# Autodesk Inventor assembly: Assembly1
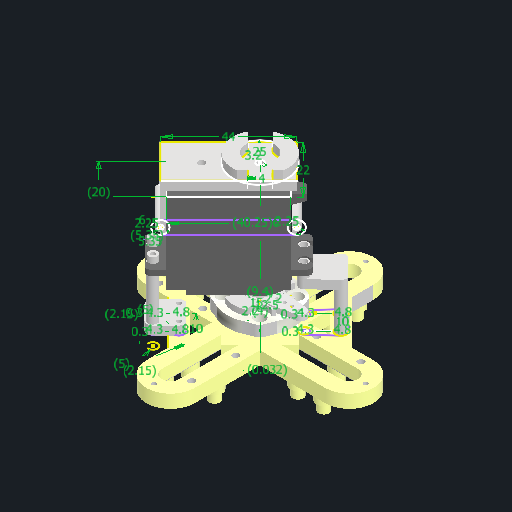
[picture p0: Inventor's stored thumbnail of the model, 512x512]
Saved by Autodesk Inventor 2026 (Build 300175000, 175)
## iProperties
Created: 2025-03-30
Part Number: Assembly1
Document SubType Name: Assembly
Designer: m_kni
Author: m_kni
## Documents named in this file (9)
- C:\Users\jerem\Desktop\Design File Archive\CAD\Gripper\Assembly1.iam
- C:\Users\jerem\Desktop\Design File Archive\CAD\Gripper\Redesign_Gripper_Baseplate.ipt
- C:\Users\jerem\Desktop\Design File Archive\CAD\Gripper\Redesign_Spinner.ipt
- C:\Users\jerem\Desktop\Design File Archive\CAD\Non 3D Printed Parts\Motors and Servos\MG 996R.ipt
- C:\Users\jerem\Desktop\Design File Archive\CAD\Non 3D Printed Parts\Motors and Servos\MG996 2 Arm Pad.ipt
- C:\Users\jerem\Desktop\Design File Archive\CAD\Gripper\gripper3leftsideservobracket.ipt
- C:\Users\jerem\Desktop\Design File Archive\CAD\Gripper\gripper3rightsideservoholder.ipt
- C:\Users\jerem\Desktop\Design File Archive\CAD\Gripper\Gripper3overhead.ipt
- C:\Users\jerem\Desktop\Design File Archive\CAD\Gripper\spinner_under.ipt
## Components (8 placed, 8 different names)
1. Redesign_Gripper_Baseplate:1 — Insert:1, Angle:1, Insert:4, Angle:2, Insert:5, Angle:3
2. Redesign_Spinner:1 — Insert:1, Insert:3, Insert:6
3. MG 996R:1 — Insert:2, Angle:1, Mate:1, Mate:2
4. MG996 2 Arm Pad:1 — Insert:2, Insert:3
5. gripper3leftsideservobracket:1 — Insert:4, Angle:2
6. gripper3rightsideservoholder:1 — Insert:5, Angle:3
7. Gripper3overhead:1 — Mate:1, Mate:2
8. spinner_under:1 — Insert:6
## Relationships (11: Insert 6, Angle 3, Mate 2)
- Insert:1: Redesign_Gripper_Baseplate:1 ↔ Redesign_Spinner:1
- Insert:2: MG 996R:1 ↔ MG996 2 Arm Pad:1
- Insert:3: Redesign_Spinner:1 ↔ MG996 2 Arm Pad:1
- Angle:1 (0 deg): Redesign_Gripper_Baseplate:1 ↔ MG 996R:1
- Insert:4: Redesign_Gripper_Baseplate:1 ↔ gripper3leftsideservobracket:1
- Angle:2 (0 deg): Redesign_Gripper_Baseplate:1 ↔ gripper3leftsideservobracket:1
- Insert:5: Redesign_Gripper_Baseplate:1 ↔ gripper3rightsideservoholder:1
- Angle:3 (0 deg): Redesign_Gripper_Baseplate:1 ↔ gripper3rightsideservoholder:1
- Mate:1: MG 996R:1 ↔ Gripper3overhead:1
- Mate:2: MG 996R:1 ↔ Gripper3overhead:1
- Insert:6: Redesign_Spinner:1 ↔ spinner_under:1
